# Autodesk Inventor assembly: Assy_wrist
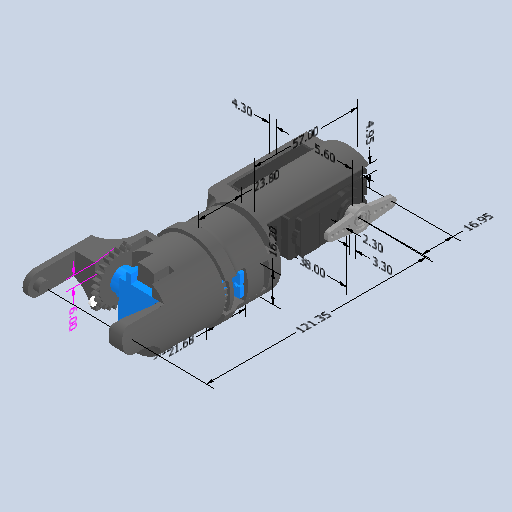
[picture p0: Inventor's stored thumbnail of the model, 512x512]
Saved by Autodesk Inventor 2024.1 (Build 281209000, 209)
## iProperties
Created: 2025-03-02
Part Number: Assy_wrist
Document SubType Name: Assembly
Designer: hibik
Author: hibik
## Documents named in this file (13)
- C:\Users\hibik\Documents\Robomech\RESCUE\ORCA\hard\arm\Assy_wrist.iam
- C:\Users\hibik\Documents\Robomech\RESCUE\ORCA\hard\arm\wrist_wrist.ipt
- C:\Users\hibik\Documents\Robomech\RESCUE\ORCA\hard\std_parts\Miusei_ms18.ipt
- C:\Users\hibik\Documents\Robomech\RESCUE\ORCA\hard\arm\hand_gear_wrist.ipt
- C:\Users\hibik\Documents\Robomech\RESCUE\ORCA\hard\std_parts\Miusei_hone_short.ipt
- C:\Users\hibik\Documents\Robomech\RESCUE\ORCA\hard\arm\wrist_hand_connector.ipt
- C:\Users\hibik\Documents\Robomech\RESCUE\ORCA\hard\arm\wrist_geard_hone.ipt
- C:\Users\hibik\Documents\Robomech\RESCUE\ORCA\hard\std_parts\bearing_6_10_3_MIR.ipt
- C:\Users\hibik\Documents\Robomech\RESCUE\ORCA\hard\arm\wrist_gear_spacer.ipt
- C:\Users\hibik\Documents\Robomech\RESCUE\ORCA\hard\arm\arm_2.ipt
- C:\Users\hibik\Documents\Robomech\RESCUE\ORCA\hard\arm\wrist_cover.ipt
- C:\Users\hibik\Documents\Robomech\RESCUE\ORCA\hard\std_parts\FS5103B.ipt
- C:\Users\hibik\Documents\Robomech\RESCUE\ORCA\hard\std_parts\feetech_servohone.ipt
## Components (15 placed, 12 different names)
1. wrist_wrist:1 — メイト:1, メイト:2, メイト:3, 挿入:3, フラッシュ:1, 挿入:6, 挿入:9
2. Miusei_ms18:1 — メイト:1, メイト:2, メイト:3, 挿入:1
3. hand_gear_wrist:1 — 挿入:2
4. Miusei_hone_short:1 — 挿入:1, 挿入:2
5. wrist_hand_connector:1 — 挿入:3, フラッシュ:1
6. Miusei_ms18:2 — 挿入:4, 角度:1, メイト:4, メイト:5, メイト:6
7. wrist_geard_hone:1 — 挿入:4, 挿入:5
8. bearing_6_10_3_MIR:1 — 挿入:5, 挿入:8
9. bearing_6_10_3_MIR:2 — 挿入:6, 挿入:7
10. wrist_gear_spacer:1 — 挿入:7, 挿入:8, 角度:1
11. arm_2:1 — メイト:4, メイト:5, メイト:6, 角度:2, メイト:7, メイト:8, メイト:9, 挿入:11
12. wrist_cover:1 — 挿入:9, 角度:2
13. FS5103B:1 — メイト:7, メイト:8, メイト:9, 挿入:10
14. feetech_servohone:1 — 挿入:10
15. bearing_6_10_3_MIR:3 — 挿入:11
## Relationships (23: Insert 11, Mate 9, Angle 2, Flush 1)
- メイト:1 [Mate]: wrist_wrist:1 ↔ Miusei_ms18:1
- メイト:2 [Mate]: wrist_wrist:1 ↔ Miusei_ms18:1
- メイト:3 [Mate]: wrist_wrist:1 ↔ Miusei_ms18:1
- 挿入:1 [Insert]: Miusei_ms18:1 ↔ Miusei_hone_short:1
- 挿入:2 [Insert]: hand_gear_wrist:1 ↔ Miusei_hone_short:1
- 挿入:3 [Insert]: wrist_wrist:1 ↔ wrist_hand_connector:1
- フラッシュ:1 [Flush]: wrist_wrist:1 ↔ wrist_hand_connector:1
- 挿入:4 [Insert]: Miusei_ms18:2 ↔ wrist_geard_hone:1
- 挿入:5 [Insert]: wrist_geard_hone:1 ↔ bearing_6_10_3_MIR:1
- 挿入:6 [Insert]: wrist_wrist:1 ↔ bearing_6_10_3_MIR:2
- 挿入:7 [Insert]: bearing_6_10_3_MIR:2 ↔ wrist_gear_spacer:1
- 挿入:8 [Insert]: bearing_6_10_3_MIR:1 ↔ wrist_gear_spacer:1
- 角度:1 [Angle] (0 deg): Miusei_ms18:2 ↔ wrist_gear_spacer:1
- メイト:4 [Mate]: Miusei_ms18:2 ↔ arm_2:1
- メイト:5 [Mate]: Miusei_ms18:2 ↔ arm_2:1
- メイト:6 [Mate]: Miusei_ms18:2 ↔ arm_2:1
- 挿入:9 [Insert] (0.5 mm): wrist_wrist:1 ↔ wrist_cover:1
- 角度:2 [Angle] (180 deg): arm_2:1 ↔ wrist_cover:1
- メイト:7 [Mate]: arm_2:1 ↔ FS5103B:1
- メイト:8 [Mate]: arm_2:1 ↔ FS5103B:1
- メイト:9 [Mate]: arm_2:1 ↔ FS5103B:1
- 挿入:10 [Insert]: FS5103B:1 ↔ feetech_servohone:1
- 挿入:11 [Insert]: arm_2:1 ↔ bearing_6_10_3_MIR:3
